# Autodesk Inventor assembly: mount3
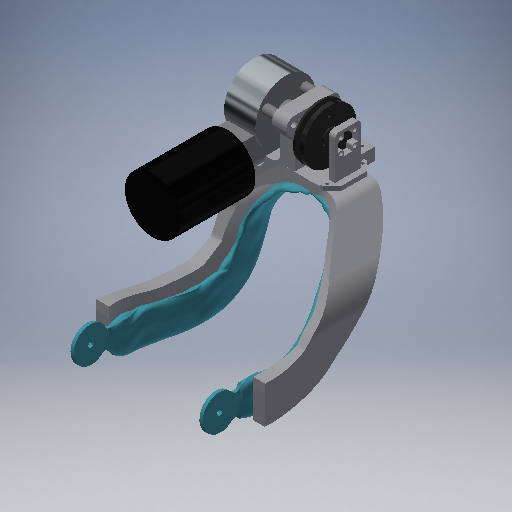
[picture p0: Inventor's stored thumbnail of the model, 512x512]
Saved by Autodesk Inventor 2025.2 (Build 292293000, 293)
## iProperties
Created: 2025-02-11
Part Number: mount3
Document SubType Name: Assembly
Designer: Alex
Author: Alex
## Documents named in this file (10)
- C:\Shared\alex-bartella-schoolwork\4tb6\4tb6-repo\CAD_Model\thigh_mount_2\thigh_mount_2\mount3.iam
- C:\Shared\alex-bartella-schoolwork\4tb6\4tb6-repo\CAD_Model\thigh_mount_2\thigh_mount_2\thigh.ipt
- C:\Shared\alex-bartella-schoolwork\4tb6\4tb6-repo\CAD_Model\thigh_mount_2\thigh_mount_2\mount3.ipt
- C:\Shared\alex-bartella-schoolwork\4tb6\4tb6-repo\CAD_Model\thigh_mount_2\thigh_mount_2\mount4.ipt
- C:\Shared\alex-bartella-schoolwork\4tb6\4tb6-repo\CAD_Model\thigh_mount_2\thigh_mount_2\motor.ipt
- C:\Shared\alex-bartella-schoolwork\4tb6\4tb6-repo\CAD_Model\thigh_mount_2\thigh_mount_2\spool_temp.ipt
- C:\Shared\alex-bartella-schoolwork\4tb6\4tb6-repo\CAD_Model\thigh_mount_2\thigh_mount_2\magnetholder.ipt
- C:\Shared\alex-bartella-schoolwork\4tb6\4tb6-repo\CAD_Model\thigh_mount_2\thigh_mount_2\imu_house_assembly.iam
- C:\Shared\alex-bartella-schoolwork\4tb6\4tb6-repo\CAD_Model\thigh_mount_2\thigh_mount_2\ANSI B18.6.7M - M6x1 x 13(6).ipt
- C:\Shared\alex-bartella-schoolwork\4tb6\4tb6-repo\CAD_Model\thigh_mount_2\thigh_mount_2\as5600mount.ipt
## Components (9 placed, 9 different names)
1. thigh:1 — Mate:1, Mate:2, Flush:1, Flush:2
2. mount3:1 — Flush:2
3. mount4:1 — Flush:4, Mate:3, Mate:4, Mate:5, Mate:12, Mate:13, Flush:5, Mate:16, Angle:1
4. motor:1 — Mate:3, Mate:4, Mate:5, Mate:6, Mate:7, Mate:8
5. spool_temp:1 — Mate:6, Mate:7, Mate:8, Mate:9, Mate:10, Mate:11
6. magnetholder:1 — Mate:9, Mate:10, Mate:11
7. imu_house_assembly:1 [sub-assembly] — Mate:12, Mate:13, Flush:5, Mate:14, Mate:15
8. Square Recessed Pan Head Machine Screw - Type III - Metric M6x1 x 13:1 — Mate:14, Mate:15
9. as5600mount:1 — Mate:16, Angle:1
## Relationships (22: Mate 16, Flush 5, Angle 1)
- Mate:1: thigh:1
- Mate:2: thigh:1
- Flush:1: thigh:1
- Flush:2: thigh:1 ↔ mount3:1
- Flush:3 (-15 mm)
- Flush:4: mount4:1
- Mate:3: mount4:1 ↔ motor:1
- Mate:4: mount4:1 ↔ motor:1
- Mate:5: mount4:1 ↔ motor:1
- Mate:6: motor:1 ↔ spool_temp:1
- Mate:7: motor:1 ↔ spool_temp:1
- Mate:8: motor:1 ↔ spool_temp:1
- Mate:9: spool_temp:1 ↔ magnetholder:1
- Mate:10: spool_temp:1 ↔ magnetholder:1
- Mate:11: spool_temp:1 ↔ magnetholder:1
- Mate:12: mount4:1 ↔ imu_house_assembly:1
- Mate:13: mount4:1 ↔ imu_house_assembly:1
- Flush:5: mount4:1 ↔ imu_house_assembly:1
- Mate:14: imu_house_assembly:1 ↔ Square Recessed Pan Head Machine Screw - Type III - Metric M6x1 x 13:1
- Mate:15: imu_house_assembly:1 ↔ Square Recessed Pan Head Machine Screw - Type III - Metric M6x1 x 13:1
- Mate:16: mount4:1 ↔ as5600mount:1
- Angle:1 (180 deg): mount4:1 ↔ as5600mount:1
